# Autodesk Inventor assembly: crane-base-assembly
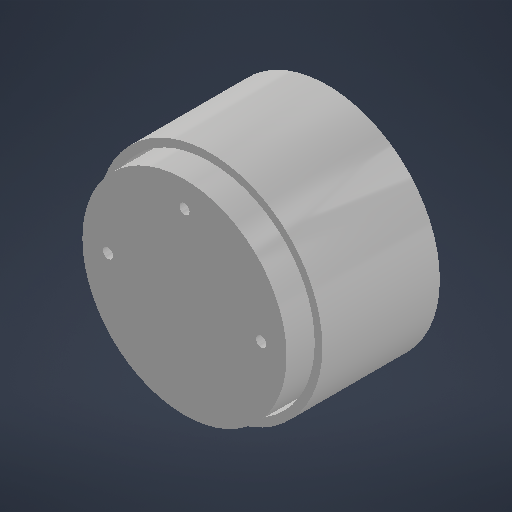
[picture p0: Inventor's stored thumbnail of the model, 512x512]
Saved by Autodesk Inventor 2026.1 (Build 301233000, 233)
## iProperties
Created: 2026-02-25
Part Number: crane-base-assembly
Document SubType Name: Assembly
Designer: dm2166
Author: dm2166
## Documents named in this file (3)
- H:\HWSYS\Desktop\Year 3\Inventor\crane-base-assembly.iam
- C:\Users\dm2166\Downloads\rotating base head.ipt
- C:\Users\dm2166\Downloads\rotating base bottom.ipt
## Components (2 placed, 2 different names)
1. rotating base head:1 — Insert:1
2. rotating base bottom:1 — Flush:1, Insert:1
## Relationships (2: Flush 1, Insert 1)
- Flush:1: rotating base bottom:1
- Insert:1: rotating base head:1 ↔ rotating base bottom:1
